# Autodesk Inventor assembly: RailMirrorIrisLensObjective
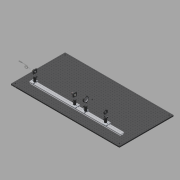
[picture p0: Inventor's stored thumbnail of the model, 180x180]
Saved by Autodesk Inventor 2018 (Build 220112000, 112)
## iProperties
Created: 2018-11-05
Part Number: RailMirrorIrisLensObjective
Document SubType Name: Assembly
Designer: Robert Campbell
Author: Robert Campbell
## Documents named in this file (10)
- \\Mac\Home\Dropbox (UCL - SWC)\work\WorkDocs\MF_BenchOptics\CAD_files\RailMirrorIrisLensObjective.iam
- \\Mac\Home\Dropbox (UCL - SWC)\work\WorkDocs\MF_BenchOptics\CAD_files\RailAndMirror.iam
- \\Mac\Home\Dropbox (UCL - SWC)\work\WorkDocs\MF_BenchOptics\CAD_files\R2_M-Step.ipt
- \\Mac\Home\Dropbox (UCL - SWC)\work\WorkDocs\MF_BenchOptics\CAD_files\LA1256-A-Solidworks.ipt
- \\Mac\Home\Dropbox (UCL - SWC)\work\WorkDocs\MF_BenchOptics\CAD_files\LM2_lensholder_on_mount.iam
- \\Mac\Home\Dropbox (UCL - SWC)\work\WorkDocs\MF_BenchOptics\CAD_files\PH50_and_carriage.iam
- \\Mac\Home\Dropbox (UCL - SWC)\work\WorkDocs\MF_BenchOptics\CAD_files\TR50_M-Solidworks.ipt
- \\Mac\Home\Dropbox (UCL - SWC)\work\WorkDocs\MF_BenchOptics\CAD_files\CP02_M-Solidworks.ipt
- \\Mac\Home\Dropbox (UCL - SWC)\work\WorkDocs\MF_BenchOptics\CAD_files\RMS4X-PF-Step.ipt
- \\Mac\Home\Dropbox (UCL - SWC)\work\WorkDocs\MF_BenchOptics\CAD_files\SM1A3-Solidworks.ipt
## Components (9 placed, 9 different names)
1. RailAndMirror:1 [sub-assembly] — Mate:1, Mate:2, Mate:5, Angle:1, Mate:14, Angle:3
2. R2_M-Step:1 — Mate:1, Mate:2
3. LA1256-A-Solidworks:1 — Mate:3, Mate:4
4. LM2_lensholder_on_mount:1 [sub-assembly] — Mate:3, Mate:4, Mate:5, Angle:1
5. PH50_and_carriage:1 [sub-assembly] — Mate:12, Mate:13, Angle:2, Mate:14, Angle:3
6. TR50_M-Solidworks:1 — Mate:10, Mate:11, Mate:12
7. CP02_M-Solidworks:1 — Mate:8, Mate:9, Mate:10, Mate:11, Mate:13, Angle:2
8. RMS4X-PF-Step:1 — Mate:6, Mate:7
9. SM1A3-Solidworks:1 — Mate:6, Mate:7, Mate:8, Mate:9
## Relationships (17: Mate 14, Angle 3)
- Mate:1: RailAndMirror:1 ↔ R2_M-Step:1
- Mate:2: RailAndMirror:1 ↔ R2_M-Step:1
- Mate:3: LA1256-A-Solidworks:1 ↔ LM2_lensholder_on_mount:1
- Mate:4: LA1256-A-Solidworks:1 ↔ LM2_lensholder_on_mount:1
- Mate:5: RailAndMirror:1 ↔ LM2_lensholder_on_mount:1
- Angle:1 (0 deg): RailAndMirror:1 ↔ LM2_lensholder_on_mount:1
- Mate:6: RMS4X-PF-Step:1 ↔ SM1A3-Solidworks:1
- Mate:7: RMS4X-PF-Step:1 ↔ SM1A3-Solidworks:1
- Mate:8: CP02_M-Solidworks:1 ↔ SM1A3-Solidworks:1
- Mate:9: CP02_M-Solidworks:1 ↔ SM1A3-Solidworks:1
- Mate:10: TR50_M-Solidworks:1 ↔ CP02_M-Solidworks:1
- Mate:11: TR50_M-Solidworks:1 ↔ CP02_M-Solidworks:1
- Mate:12: PH50_and_carriage:1 ↔ TR50_M-Solidworks:1
- Mate:13 (26 mm): PH50_and_carriage:1 ↔ CP02_M-Solidworks:1
- Angle:2 (0 deg): PH50_and_carriage:1 ↔ CP02_M-Solidworks:1
- Mate:14: RailAndMirror:1 ↔ PH50_and_carriage:1
- Angle:3 (0 deg): RailAndMirror:1 ↔ PH50_and_carriage:1
